# Autodesk Inventor assembly: EndAssembly
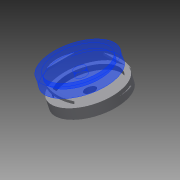
[picture p0: Inventor's stored thumbnail of the model, 180x180]
Saved by Autodesk Inventor 2014 (Build 180170000, 170)
## iProperties
Created: 2013-05-26
Part Number: EndAssembly
Document SubType Name: Assembly
Designer: Felix
Author: Felix
## Documents named in this file (3)
- C:\Users\Felix\Desktop\Beep\Hardware\Z132053\EndAssembly.iam
- C:\Users\Felix\Desktop\Beep\Hardware\Z132053\snap.ipt
- C:\Users\Felix\Desktop\Beep\Hardware\Z132053\EndCap.ipt
## Components (2 placed, 2 different names)
1. snap:1 — Mate:1, Mate:3
2. EndCap:1 — Mate:2, Mate:3
## Relationships (3: Mate 3)
- Mate:1: snap:1
- Mate:2: EndCap:1
- Mate:3: snap:1 ↔ EndCap:1
